# Autodesk Inventor assembly: Vacubot v1
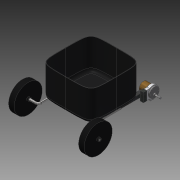
[picture p0: Inventor's stored thumbnail of the model, 180x180]
Saved by Autodesk Inventor 2014 SP1 (Build 180222100, 222)
## iProperties
Created: 2013-12-26
Part Number: Vacubot v1
Document SubType Name: Assembly
Designer: tom
Author: tom
## Documents named in this file (8)
- C:\Users\tom\Documents\GitHub\Vacubot\Inventor\Vacubot v1.iam
- C:\Users\tom\Documents\GitHub\Vacubot\Inventor\Base.ipt
- C:\Users\tom\Documents\GitHub\Vacubot\Inventor\Base Plate.ipt
- C:\Users\tom\Documents\GitHub\Vacubot\Inventor\Motor Mount.ipt
- C:\Users\tom\Documents\GitHub\Vacubot\Inventor\Wheel Original.iam
- C:\Users\tom\Documents\GitHub\Vacubot\Inventor\Motor Mount_MIR.ipt
- C:\Users\tom\Documents\GitHub\Vacubot\Inventor\Wheel Original_MIR.iam
- C:\Users\tom\Documents\GitHub\Vacubot\Inventor\Drive Motor.ipt
## Components (7 placed, 7 different names)
1. Chassis — Mate:4, Mate:6, Mate:7
2. Base Plate:1
3. Motor Mount:1 — Mate:4, Mate:6, Mate:7, Mate:8, Flush:1
4. Wheel Original:1 [sub-assembly]
5. Motor Mount_MIR:1
6. Wheel Original_MIR:1 [sub-assembly]
7. Drive Motor:1 — Mate:8, Flush:1
## Relationships (8: Mate 6, Tangent 1, Flush 1)
- [Mate] (-6.35 mm): Wheel Original:1
- [Tangent]: Chassis ↔ Wheel Original:1
- [Mate] (-6.35 mm): Wheel Original:1
- Mate:4: Chassis ↔ Motor Mount:1
- Mate:6 (1.988 mm): Chassis ↔ Motor Mount:1
- Mate:7: Chassis ↔ Motor Mount:1
- Mate:8: Motor Mount:1 ↔ Drive Motor:1
- Flush:1 (-5 mm): Motor Mount:1 ↔ Drive Motor:1
